# Autodesk Inventor assembly: FarmBot
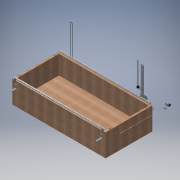
[picture p0: Inventor's stored thumbnail of the model, 180x180]
Saved by Autodesk Inventor 2017 (Build 210142000, 142)
## iProperties
Created: 2016-12-12
Part Number: FarmBot
Document SubType Name: Assembly
Designer: umr
Author: umr
## Documents named in this file (9)
- D:\SeniorProject\Models2\FarmBot.iam
- D:\SeniorProject\Models2\BedAssembly\BedAseembly.iam
- D:\SeniorProject\Models2\Case\Case.iam
- D:\SeniorProject\Models2\LED Structure\LED Structure Assembly.iam
- D:\SeniorProject\Models2\Gantry\GantryDown.iam
- D:\SeniorProject\Models2\BeltMain.ipt
- D:\SeniorProject\Models2\WheelAssembly\OurWheelAssemblyBig.iam
- D:\SeniorProject\Models2\WheelAssembly\OurWheelAssembly.iam
- D:\SeniorProject\Models2\LBent_PScrew.ipt
## Components (8 placed, 8 different names)
1. BedAseembly:2 [sub-assembly] — Mate:10, Mate:11, Mate:12, Mate:13, Mate:14, Mate:15, Mate:16, Mate:18, Flush:1, Mate:19, Mate:20, Tangent:2, Tangent:3
2. Case:1 [sub-assembly] — Mate:10, Mate:11, Mate:12, Mate:13
3. LED Structure Assembly:1 [sub-assembly] — Mate:14, Mate:15, Mate:16
4. GantryDown:1 [sub-assembly] — Mate:18, Flush:1, Tangent:1, Mate:22, Mate:23, Tangent:4
5. BeltMain:1 — Mate:19, Mate:20, Tangent:1
6. OurWheelAssemblyBig:1 [sub-assembly] — Mate:22, Tangent:2, Tangent:5
7. OurWheelAssembly:1 [sub-assembly] — Tangent:3, Mate:23
8. LBent_PScrew:1 — Tangent:4, Tangent:5
## Relationships (18: Mate 12, Tangent 5, Flush 1)
- Mate:10: BedAseembly:2 ↔ Case:1
- Mate:11: BedAseembly:2 ↔ Case:1
- Mate:12: BedAseembly:2 ↔ Case:1
- Mate:13: BedAseembly:2 ↔ Case:1
- Mate:14: BedAseembly:2 ↔ LED Structure Assembly:1
- Mate:15: BedAseembly:2 ↔ LED Structure Assembly:1
- Mate:16: BedAseembly:2 ↔ LED Structure Assembly:1
- Mate:18: BedAseembly:2 ↔ GantryDown:1
- Flush:1 (100 mm): BedAseembly:2 ↔ GantryDown:1
- Mate:19: BedAseembly:2 ↔ BeltMain:1
- Mate:20 (3 mm): BedAseembly:2 ↔ BeltMain:1
- Tangent:1: GantryDown:1 ↔ BeltMain:1
- Mate:22: GantryDown:1 ↔ OurWheelAssemblyBig:1
- Tangent:2: BedAseembly:2 ↔ OurWheelAssemblyBig:1
- Tangent:3: BedAseembly:2 ↔ OurWheelAssembly:1
- Mate:23: GantryDown:1 ↔ OurWheelAssembly:1
- Tangent:4: GantryDown:1 ↔ LBent_PScrew:1
- Tangent:5 (1.5 mm): OurWheelAssemblyBig:1 ↔ LBent_PScrew:1
